# Autodesk Inventor assembly: dish
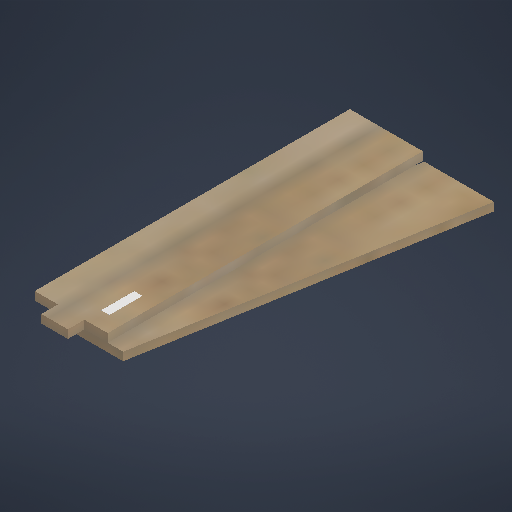
[picture p0: Inventor's stored thumbnail of the model, 512x512]
Saved by Autodesk Inventor 2026.1 (Build 301233020, 233B)
## iProperties
Created: 2025-09-27
Part Number: dish
Document SubType Name: Assembly
Designer: hibik
Author: hibik
## Documents named in this file (4)
- C:\Users\hibik\Documents\Robomech\conveyer\belt\dish.iam
- C:\Users\hibik\Documents\Robomech\conveyer\belt\dish_upper.ipt
- C:\Users\hibik\Documents\Robomech\conveyer\belt\dish_under.ipt
- C:\Users\hibik\Documents\Robomech\conveyer\belt\tab.ipt
## Components (3 placed, 3 different names)
1. dish_upper:1 — メイト:1, フラッシュ:1, フラッシュ:2, フラッシュ:3, メイト:2, メイト:3
2. dish_under:1 — メイト:1, フラッシュ:1, フラッシュ:2
3. tab:1 — フラッシュ:3, メイト:2, メイト:3
## Relationships (6: Mate 3, Flush 3)
- メイト:1 [Mate]: dish_upper:1 ↔ dish_under:1
- フラッシュ:1 [Flush]: dish_upper:1 ↔ dish_under:1
- フラッシュ:2 [Flush]: dish_upper:1 ↔ dish_under:1
- フラッシュ:3 [Flush]: dish_upper:1 ↔ tab:1
- メイト:2 [Mate]: dish_upper:1 ↔ tab:1
- メイト:3 [Mate]: dish_upper:1 ↔ tab:1
